# Autodesk Inventor assembly: Assembly
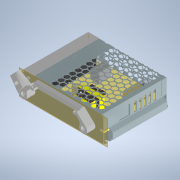
[picture p0: Inventor's stored thumbnail of the model, 180x180]
Saved by Autodesk Inventor 2021 (Build 250183000, 183)
## iProperties
Created: 2020-10-20
Part Number: Assembly
Document SubType Name: Assembly
Designer: VM
Author: VM
## Documents named in this file (5)
- \\vmware-host\Shared Folders\Documents\Projects Stuff\wakeuplamp\CAD\Assembly.iam
- \\vmware-host\Shared Folders\Documents\Projects Stuff\wakeuplamp\CAD\LRS-50-Series(MW).ipt
- \\vmware-host\Shared Folders\Documents\Projects Stuff\wakeuplamp\CAD\Main.ipt
- \\vmware-host\Shared Folders\Documents\Projects Stuff\wakeuplamp\CAD\Part7.ipt
- \\vmware-host\Shared Folders\Documents\Projects Stuff\wakeuplamp\CAD\Hangar.ipt
## Components (4 placed, 4 different names)
1. LRS-50-Series(MW):1 — Mate:1, Mate:2, Mate:3, Flush:4, Flush:5, Mate:5, Mate:6, Mate:7
2. Main:1 — Mate:1, Mate:2, Mate:3
3. Part7:1 — Flush:4, Flush:5, Mate:4, Mate:6, Mate:7
4. Hangar:1 — Mate:4, Mate:5
## Relationships (9: Mate 7, Flush 2)
- Mate:1: LRS-50-Series(MW):1 ↔ Main:1
- Mate:2: LRS-50-Series(MW):1 ↔ Main:1
- Mate:3: LRS-50-Series(MW):1 ↔ Main:1
- Flush:4: LRS-50-Series(MW):1 ↔ Part7:1
- Flush:5: LRS-50-Series(MW):1 ↔ Part7:1
- Mate:4: Part7:1 ↔ Hangar:1
- Mate:5: LRS-50-Series(MW):1 ↔ Hangar:1
- Mate:6: LRS-50-Series(MW):1 ↔ Part7:1
- Mate:7: LRS-50-Series(MW):1 ↔ Part7:1
